# Autodesk Inventor assembly: DriveTrainBase
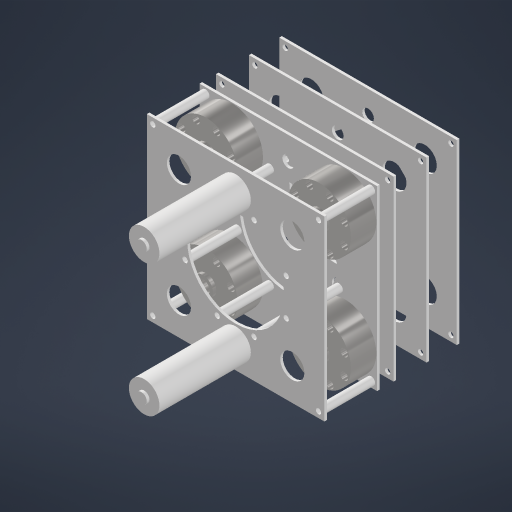
[picture p0: Inventor's stored thumbnail of the model, 512x512]
Saved by Autodesk Inventor 2024 (Build 280153000, 153)
## iProperties
Created: 2025-02-12
Part Number: DriveTrainBase
Document SubType Name: Assembly
Designer: Tommy Rohmann
Author: Tommy Rohmann
## Documents named in this file (9)
- C:\Users\Tommy Rohmann\OneDrive\Projects\Microgravity-Press-Washing-Machine\System Design and Documentation\Inventor Design Project\DriveTrainBase.iam
- C:\Users\Tommy Rohmann\OneDrive\Projects\Microgravity-Press-Washing-Machine\System Design and Documentation\Inventor Design Project\LoadCellBase.ipt
- C:\Users\Tommy Rohmann\OneDrive\Projects\Microgravity-Press-Washing-Machine\System Design and Documentation\Inventor Design Project\LoadCell.ipt
- C:\Users\Tommy Rohmann\OneDrive\Projects\Microgravity-Press-Washing-Machine\System Design and Documentation\Inventor Design Project\DriveMotor.ipt
- C:\Users\Tommy Rohmann\OneDrive\Projects\Microgravity-Press-Washing-Machine\System Design and Documentation\Inventor Design Project\SUBDriveShaftACME.iam
- C:\Users\Tommy Rohmann\OneDrive\Projects\Microgravity-Press-Washing-Machine\System Design and Documentation\Inventor Design Project\TopBase.ipt
- C:\Users\Tommy Rohmann\OneDrive\Projects\Microgravity-Press-Washing-Machine\System Design and Documentation\Inventor Design Project\LAYOUT.ipt
- C:\Users\Tommy Rohmann\OneDrive\Projects\Microgravity-Press-Washing-Machine\System Design and Documentation\Inventor Design Project\DriveTrainBaseSpacer.ipt
- C:\Users\Tommy Rohmann\OneDrive\Projects\Microgravity-Press-Washing-Machine\System Design and Documentation\Inventor Design Project\ChainBase.ipt
## Components (25 placed, 8 different names)
1. LoadCellBase:1 — Mate:1, Mate:2, Mate:3, Mate:4, Mate:5, Mate:6, Mate:7, Mate:8, Mate:9, Mate:10, Mate:11, Mate:12, Mate:22, Mate:23, Mate:24, Mate:25, Mate:26, Mate:27, Mate:28, Mate:29, Mate:30, Mate:31, Mate:32, Mate:38, Mate:45
2. LoadCell:1 — Mate:1, Mate:7, Mate:12, Mate:13, Mate:14
3. LoadCell:2 — Mate:4, Mate:6, Mate:11
4. LoadCell:3 — Mate:3, Mate:5, Mate:10
5. LoadCell:4 — Mate:2, Mate:8, Mate:9
6. DriveMotor:1 — Mate:20, Mate:21
7. SUBDriveShaftACME:1 [sub-assembly] — Mate:13, Mate:14, Mate:15, Mate:16, Mate:49, Mate:50, Mate:51, Mate:53, Mate:54, Mate:55
8. LAYOUT:1
9. TopBase:1 — Mate:15, Mate:16, Mate:18, Mate:19, Mate:20, Mate:21, Mate:22, Mate:33, Mate:34, Mate:35, Mate:36, Mate:37, Mate:39, Mate:40, Mate:41, Mate:42, Mate:43, Mate:44, Mate:46, Mate:47, Mate:48, Mate:52
10. DriveMotor:3 — Mate:18, Mate:19
11. DriveTrainBaseSpacer:1 — Mate:23, Mate:37
12. DriveTrainBaseSpacer:2 — Mate:30, Mate:40
13. DriveTrainBaseSpacer:3 — Mate:31, Mate:43
14. DriveTrainBaseSpacer:4 — Mate:29, Mate:44
15. DriveTrainBaseSpacer:5 — Mate:32, Mate:33
16. DriveTrainBaseSpacer:6 — Mate:38, Mate:39
17. DriveTrainBaseSpacer:7 — Mate:28, Mate:34
18. DriveTrainBaseSpacer:8 — Mate:27, Mate:42
19. DriveTrainBaseSpacer:9 — Mate:26, Mate:41
20. DriveTrainBaseSpacer:10 — Mate:25, Mate:36
21. DriveTrainBaseSpacer:11 — Mate:24, Mate:35
22. DriveTrainBaseSpacer:12 — Mate:45, Mate:46
23. ChainBase:1 — Mate:47, Mate:50, Mate:55
24. ChainBase:2 — Mate:48, Mate:49, Mate:51
25. ChainBase:3 — Mate:52, Mate:53, Mate:54
## Relationships (54: Mate 54)
- Mate:1: LoadCellBase:1 ↔ LoadCell:1
- Mate:2: LoadCellBase:1 ↔ LoadCell:4
- Mate:3: LoadCellBase:1 ↔ LoadCell:3
- Mate:4: LoadCellBase:1 ↔ LoadCell:2
- Mate:5: LoadCellBase:1 ↔ LoadCell:3
- Mate:6: LoadCellBase:1 ↔ LoadCell:2
- Mate:7: LoadCellBase:1 ↔ LoadCell:1
- Mate:8: LoadCellBase:1 ↔ LoadCell:4
- Mate:9: LoadCellBase:1 ↔ LoadCell:4
- Mate:10: LoadCellBase:1 ↔ LoadCell:3
- Mate:11: LoadCellBase:1 ↔ LoadCell:2
- Mate:12: LoadCellBase:1 ↔ LoadCell:1
- Mate:13: LoadCell:1 ↔ SUBDriveShaftACME:1
- Mate:14: LoadCell:1 ↔ SUBDriveShaftACME:1
- Mate:15: SUBDriveShaftACME:1 ↔ TopBase:1
- Mate:16: SUBDriveShaftACME:1 ↔ TopBase:1
- Mate:18: TopBase:1 ↔ DriveMotor:3
- Mate:19: TopBase:1 ↔ DriveMotor:3
- Mate:20: DriveMotor:1 ↔ TopBase:1
- Mate:21: DriveMotor:1 ↔ TopBase:1
- Mate:22: LoadCellBase:1 ↔ TopBase:1
- Mate:23: LoadCellBase:1 ↔ DriveTrainBaseSpacer:1
- Mate:24: LoadCellBase:1 ↔ DriveTrainBaseSpacer:11
- Mate:25: LoadCellBase:1 ↔ DriveTrainBaseSpacer:10
- Mate:26: LoadCellBase:1 ↔ DriveTrainBaseSpacer:9
- Mate:27: LoadCellBase:1 ↔ DriveTrainBaseSpacer:8
- Mate:28: LoadCellBase:1 ↔ DriveTrainBaseSpacer:7
- Mate:29: LoadCellBase:1 ↔ DriveTrainBaseSpacer:4
- Mate:30: LoadCellBase:1 ↔ DriveTrainBaseSpacer:2
- Mate:31: LoadCellBase:1 ↔ DriveTrainBaseSpacer:3
- Mate:32: LoadCellBase:1 ↔ DriveTrainBaseSpacer:5
- Mate:33: TopBase:1 ↔ DriveTrainBaseSpacer:5
- Mate:34: TopBase:1 ↔ DriveTrainBaseSpacer:7
- Mate:35: TopBase:1 ↔ DriveTrainBaseSpacer:11
- Mate:36: TopBase:1 ↔ DriveTrainBaseSpacer:10
- Mate:37: TopBase:1 ↔ DriveTrainBaseSpacer:1
- Mate:38: LoadCellBase:1 ↔ DriveTrainBaseSpacer:6
- Mate:39: TopBase:1 ↔ DriveTrainBaseSpacer:6
- Mate:40: TopBase:1 ↔ DriveTrainBaseSpacer:2
- Mate:41: TopBase:1 ↔ DriveTrainBaseSpacer:9
- Mate:42: TopBase:1 ↔ DriveTrainBaseSpacer:8
- Mate:43: TopBase:1 ↔ DriveTrainBaseSpacer:3
- Mate:44: TopBase:1 ↔ DriveTrainBaseSpacer:4
- Mate:45: LoadCellBase:1 ↔ DriveTrainBaseSpacer:12
- Mate:46: TopBase:1 ↔ DriveTrainBaseSpacer:12
- Mate:47: TopBase:1 ↔ ChainBase:1
- Mate:48: TopBase:1 ↔ ChainBase:2
- Mate:49: SUBDriveShaftACME:1 ↔ ChainBase:2
- Mate:50: SUBDriveShaftACME:1 ↔ ChainBase:1
- Mate:51: SUBDriveShaftACME:1 ↔ ChainBase:2
- Mate:52: TopBase:1 ↔ ChainBase:3
- Mate:53: SUBDriveShaftACME:1 ↔ ChainBase:3
- Mate:54: SUBDriveShaftACME:1 ↔ ChainBase:3
- Mate:55: SUBDriveShaftACME:1 ↔ ChainBase:1
